# Autodesk Inventor assembly: Setup_1
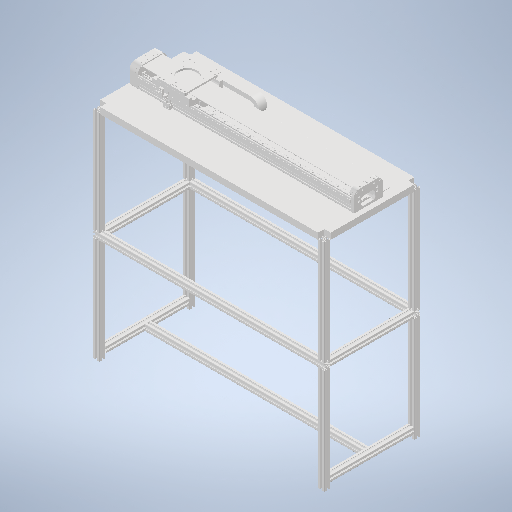
[picture p0: Inventor's stored thumbnail of the model, 512x512]
Saved by Autodesk Inventor 2025 (Build 290162000, 162)
## iProperties
Created: 2024-06-18
Part Number: Setup_1
Document SubType Name: Assembly
Designer: User
Author: User
## Documents named in this file (8)
- C:\Users\User\OneDrive\Documents\FYP\Inventor_Designs\Metal Profile\Setup_1.iam
- C:\Users\User\OneDrive\Documents\FYP\Inventor_Designs\Metal Profile\Metal Profile 110 cm.ipt
- C:\Users\User\OneDrive\Documents\FYP\Inventor_Designs\Metal Profile\Metal Profile 40 cm.ipt
- C:\Users\User\OneDrive\Documents\FYP\Inventor_Designs\Metal Profile\Metal Profile 50 cm.ipt
- C:\Users\User\OneDrive\Documents\FYP\Inventor_Designs\Metal Profile\Metal Profile 104 cm.ipt
- C:\Users\User\OneDrive\Documents\FYP\Inventor_Designs\Linear Motor\Motor.ipt
- C:\Users\User\OneDrive\Documents\FYP\Inventor_Designs\Designs_Arm\Platform.ipt
- C:\Users\User\OneDrive\Documents\FYP\Inventor_Designs\Platform\Platform_Arm.ipt
## Components (18 placed, 7 different names)
1. Metal Profile 110 cm:1 — Mate:1, Mate:3, Flush:1, Mate:4, Flush:3, Mate:6, Mate:7, Mate:8, Flush:5, Mate:15, Mate:16, Mate:17, Mate:57, Mate:58
2. Metal Profile 40 cm:2 — Mate:1, Mate:2, Mate:3, Flush:1, Flush:2, Flush:3, Mate:6, Mate:23
3. Metal Profile 110 cm:2 — Mate:2, Flush:2, Mate:5, Flush:4, Mate:9, Mate:10, Mate:11, Mate:12, Mate:13, Mate:14, Mate:47, Mate:56, Mate:61
4. Metal Profile 40 cm:3 — Mate:4, Mate:5, Flush:4, Mate:20
5. Metal Profile 50 cm:1 — Mate:7, Mate:8, Flush:5, Mate:22, Mate:50, Mate:51
6. Metal Profile 50 cm:2 — Mate:9, Mate:10, Mate:11, Mate:21, Mate:48, Mate:49
7. Metal Profile 50 cm:3 — Mate:15, Mate:16, Mate:17, Mate:18, Mate:52, Mate:53
8. Metal Profile 50 cm:4 — Mate:12, Mate:13, Mate:14, Mate:19, Mate:54, Mate:55
9. Metal Profile 40 cm:4 — Mate:18, Mate:19, Mate:20, Mate:59, Mate:60
10. Metal Profile 40 cm:5 — Mate:21, Mate:22, Mate:23
11. Metal Profile 50 cm:5 — Mate:50, Mate:51, Mate:58
12. Metal Profile 50 cm:6 — Mate:47, Mate:48, Mate:49
13. Metal Profile 50 cm:7 — Mate:52, Mate:53, Mate:57
14. Metal Profile 50 cm:8 — Mate:54, Mate:55, Mate:56, Mate:62, Mate:63
15. Metal Profile 104 cm:1 — Mate:59, Mate:60, Mate:61
16. Motor:1 — Mate:64, Flush:6, Flush:7
17. Platform:1
18. Platform_Arm:1 — Mate:62, Mate:63, Mate:64, Flush:6, Flush:7
## Relationships (48: Mate 41, Flush 7)
- Mate:1: Metal Profile 110 cm:1 ↔ Metal Profile 40 cm:2
- Mate:2: Metal Profile 40 cm:2 ↔ Metal Profile 110 cm:2
- Mate:3: Metal Profile 110 cm:1 ↔ Metal Profile 40 cm:2
- Flush:1: Metal Profile 110 cm:1 ↔ Metal Profile 40 cm:2
- Flush:2: Metal Profile 40 cm:2 ↔ Metal Profile 110 cm:2
- Mate:4: Metal Profile 110 cm:1 ↔ Metal Profile 40 cm:3
- Flush:3: Metal Profile 110 cm:1 ↔ Metal Profile 40 cm:2
- Mate:5: Metal Profile 110 cm:2 ↔ Metal Profile 40 cm:3
- Flush:4: Metal Profile 110 cm:2 ↔ Metal Profile 40 cm:3
- Mate:6: Metal Profile 110 cm:1 ↔ Metal Profile 40 cm:2
- Mate:7: Metal Profile 110 cm:1 ↔ Metal Profile 50 cm:1
- Mate:8: Metal Profile 110 cm:1 ↔ Metal Profile 50 cm:1
- Flush:5: Metal Profile 110 cm:1 ↔ Metal Profile 50 cm:1
- Mate:9: Metal Profile 110 cm:2 ↔ Metal Profile 50 cm:2
- Mate:10: Metal Profile 110 cm:2 ↔ Metal Profile 50 cm:2
- Mate:11: Metal Profile 110 cm:2 ↔ Metal Profile 50 cm:2
- Mate:12: Metal Profile 110 cm:2 ↔ Metal Profile 50 cm:4
- Mate:13: Metal Profile 110 cm:2 ↔ Metal Profile 50 cm:4
- Mate:14: Metal Profile 110 cm:2 ↔ Metal Profile 50 cm:4
- Mate:15: Metal Profile 110 cm:1 ↔ Metal Profile 50 cm:3
- Mate:16: Metal Profile 110 cm:1 ↔ Metal Profile 50 cm:3
- Mate:17: Metal Profile 110 cm:1 ↔ Metal Profile 50 cm:3
- Mate:18: Metal Profile 50 cm:3 ↔ Metal Profile 40 cm:4
- Mate:19: Metal Profile 50 cm:4 ↔ Metal Profile 40 cm:4
- Mate:20 (450 mm): Metal Profile 40 cm:3 ↔ Metal Profile 40 cm:4
- Mate:21: Metal Profile 50 cm:2 ↔ Metal Profile 40 cm:5
- Mate:22: Metal Profile 50 cm:1 ↔ Metal Profile 40 cm:5
- Mate:23 (450 mm): Metal Profile 40 cm:2 ↔ Metal Profile 40 cm:5
- Mate:47: Metal Profile 110 cm:2 ↔ Metal Profile 50 cm:6
- Mate:48: Metal Profile 50 cm:2 ↔ Metal Profile 50 cm:6
- Mate:49: Metal Profile 50 cm:2 ↔ Metal Profile 50 cm:6
- Mate:50: Metal Profile 50 cm:1 ↔ Metal Profile 50 cm:5
- Mate:51: Metal Profile 50 cm:1 ↔ Metal Profile 50 cm:5
- Mate:52: Metal Profile 50 cm:3 ↔ Metal Profile 50 cm:7
- Mate:53: Metal Profile 50 cm:3 ↔ Metal Profile 50 cm:7
- Mate:54: Metal Profile 50 cm:4 ↔ Metal Profile 50 cm:8
- Mate:55: Metal Profile 50 cm:4 ↔ Metal Profile 50 cm:8
- Mate:56: Metal Profile 110 cm:2 ↔ Metal Profile 50 cm:8
- Mate:57: Metal Profile 110 cm:1 ↔ Metal Profile 50 cm:7
- Mate:58: Metal Profile 110 cm:1 ↔ Metal Profile 50 cm:5
- Mate:59 (185 mm): Metal Profile 40 cm:4 ↔ Metal Profile 104 cm:1
- Mate:60: Metal Profile 40 cm:4 ↔ Metal Profile 104 cm:1
- Mate:61 (499 mm): Metal Profile 110 cm:2 ↔ Metal Profile 104 cm:1
- Mate:62: Metal Profile 50 cm:8 ↔ Platform_Arm:1
- Mate:63: Metal Profile 50 cm:8 ↔ Platform_Arm:1
- Mate:64: Motor:1 ↔ Platform_Arm:1
- Flush:6 (20 mm): Motor:1 ↔ Platform_Arm:1
- Flush:7 (160 mm): Motor:1 ↔ Platform_Arm:1
